# Autodesk Inventor assembly: Conexão
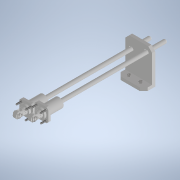
[picture p0: Inventor's stored thumbnail of the model, 180x180]
Saved by Autodesk Inventor 2021 (Build 250183000, 183)
## iProperties
Created: 2021-07-23
Part Number: Conexão
Document SubType Name: Assembly
Designer: Giovanni
Author: Giovanni
## Documents named in this file (9)
- C:\Users\irineu\Documents\Inventor\MotorRadial7\Conexão.iam
- C:\Users\irineu\Documents\Inventor\MotorRadial7\Peça28.ipt
- C:\Users\irineu\Documents\Inventor\MotorRadial7\Peça17.ipt
- C:\Users\irineu\Documents\Inventor\MotorRadial7\Peça32.ipt
- C:\Users\irineu\Documents\Inventor\MotorRadial7\Peça29.ipt
- C:\Users\irineu\Documents\Inventor\MotorRadial7\Peça30.ipt
- C:\Users\irineu\Documents\Inventor\MotorRadial7\Peça31.ipt
- C:\Users\irineu\Documents\Inventor\Content Center Files\R2021\pt-BR\DIN 6799\DIN 6799 - 5 6.ipt
- C:\Users\irineu\Documents\Inventor\Content Center Files\R2021\pt-BR\DIN 912\DIN 912 - M4 x 0,7 x 16 x 14,25.ipt
## Components (25 placed, 8 different names)
1. Peça28:1 — Alinhado:1, Coincidente:1, Coincidente:2, Coincidente:6, Coincidente:9, Coincidente:13, Inserir:9, Coincidente:22, Inserir:10, Inserir:11
2. Peça28:2 — Alinhado:1, Alinhado:2, Alinhado:3, Coincidente:3, Coincidente:4, Coincidente:8, Coincidente:10, Inserir:5, Inserir:6, Inserir:7, Inserir:8
3. Peça17:1 — Coincidente:1, Coincidente:2, Coincidente:5
4. Peça17:2 — Coincidente:3, Coincidente:4, Coincidente:7
5. Peça32:1 — Coincidente:5, Coincidente:6, Coincidente:9, Coincidente:11, Coincidente:16, Coincidente:17
6. Peça32:2 — Coincidente:7, Coincidente:8, Coincidente:10, Coincidente:12, Coincidente:14, Coincidente:15
7. Peça29:1 — Coincidente:11, Coincidente:12, Ângulo:1, Coincidente:13, Inserir:12
8. Peça30:1 — Coincidente:14, Coincidente:15, Coincidente:20, Coincidente:21, Inserir:2, Inserir:4
9. Peça30:2 — Coincidente:16, Coincidente:17, Coincidente:18, Coincidente:19, Inserir:1, Inserir:3
10. Peça31:1 — Coincidente:18, Coincidente:19
11. Peça31:2 — Coincidente:20, Coincidente:21
12. DIN 6799 5:1 — Inserir:2
13. DIN 6799 5:2 — Inserir:1
14. DIN 6799 5:3 — Inserir:3
15. DIN 6799 5:4 — Inserir:4
16. DIN 912 - substituído por DIN EN ISO 4762 M4 x 16:1 — Inserir:5
17. DIN 912 - substituído por DIN EN ISO 4762 M4 x 16:2 — Inserir:6
18. DIN 912 - substituído por DIN EN ISO 4762 M4 x 16:3 — Inserir:8
19. DIN 912 - substituído por DIN EN ISO 4762 M4 x 16:4 — Inserir:7
20. DIN 912 - substituído por DIN EN ISO 4762 M4 x 16:5 — Inserir:9
21. DIN 912 - substituído por DIN EN ISO 4762 M4 x 16:6 — Inserir:10
22. DIN 912 - substituído por DIN EN ISO 4762 M4 x 16:7 — Inserir:11
23. DIN 912 - substituído por DIN EN ISO 4762 M4 x 16:8 — Coincidente:22
24. DIN 912 - substituído por DIN EN ISO 4762 M4 x 16:9 — Inserir:12
25. DIN 912 - substituído por DIN EN ISO 4762 M4 x 16:10
## Component patterns: (2 elements, first: DIN 912 - substituído por DIN EN ISO 4762 M4 x 16:9)
## Relationships (38: Mate 22, Insert 12, Flush 3, Angle 1)
- Alinhado:1 [Flush]: Peça28:1 ↔ Peça28:2
- Alinhado:2 [Flush] (40 mm): Peça28:2
- Alinhado:3 [Flush] (13 mm): Peça28:2
- Coincidente:1 [Mate]: Peça28:1 ↔ Peça17:1
- Coincidente:2 [Mate]: Peça28:1 ↔ Peça17:1
- Coincidente:3 [Mate]: Peça28:2 ↔ Peça17:2
- Coincidente:4 [Mate]: Peça28:2 ↔ Peça17:2
- Coincidente:5 [Mate]: Peça17:1 ↔ Peça32:1
- Coincidente:6 [Mate]: Peça28:1 ↔ Peça32:1
- Coincidente:7 [Mate]: Peça17:2 ↔ Peça32:2
- Coincidente:8 [Mate]: Peça28:2 ↔ Peça32:2
- Coincidente:9 [Mate]: Peça28:1 ↔ Peça32:1
- Coincidente:10 [Mate]: Peça28:2 ↔ Peça32:2
- Coincidente:11 [Mate]: Peça32:1 ↔ Peça29:1
- Coincidente:12 [Mate]: Peça32:2 ↔ Peça29:1
- Ângulo:1 [Angle] (0 deg): Peça29:1
- Coincidente:13 [Mate] (267.5 mm): Peça28:1 ↔ Peça29:1
- Coincidente:14 [Mate]: Peça32:2 ↔ Peça30:1
- Coincidente:15 [Mate]: Peça32:2 ↔ Peça30:1
- Coincidente:16 [Mate]: Peça32:1 ↔ Peça30:2
- Coincidente:17 [Mate]: Peça32:1 ↔ Peça30:2
- Coincidente:18 [Mate]: Peça30:2 ↔ Peça31:1
- Coincidente:19 [Mate]: Peça30:2 ↔ Peça31:1
- Coincidente:20 [Mate]: Peça30:1 ↔ Peça31:2
- Coincidente:21 [Mate]: Peça30:1 ↔ Peça31:2
- Inserir:1: Peça30:2 ↔ DIN 6799 5:2
- Inserir:2: Peça30:1 ↔ DIN 6799 5:1
- Inserir:3: Peça30:2 ↔ DIN 6799 5:3
- Inserir:4: Peça30:1 ↔ DIN 6799 5:4
- Inserir:5: Peça28:2 ↔ DIN 912 - substituído por DIN EN ISO 4762 M4 x 16:1
- Inserir:6: Peça28:2 ↔ DIN 912 - substituído por DIN EN ISO 4762 M4 x 16:2
- Inserir:7: Peça28:2 ↔ DIN 912 - substituído por DIN EN ISO 4762 M4 x 16:4
- Inserir:8: Peça28:2 ↔ DIN 912 - substituído por DIN EN ISO 4762 M4 x 16:3
- Inserir:9: Peça28:1 ↔ DIN 912 - substituído por DIN EN ISO 4762 M4 x 16:5
- Coincidente:22 [Mate]: Peça28:1 ↔ DIN 912 - substituído por DIN EN ISO 4762 M4 x 16:8
- Inserir:10: Peça28:1 ↔ DIN 912 - substituído por DIN EN ISO 4762 M4 x 16:6
- Inserir:11: Peça28:1 ↔ DIN 912 - substituído por DIN EN ISO 4762 M4 x 16:7
- Inserir:12: Peça29:1 ↔ DIN 912 - substituído por DIN EN ISO 4762 M4 x 16:9
